# Autodesk Inventor assembly: Assembly1
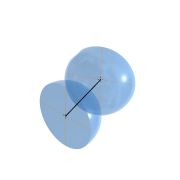
[picture p0: Inventor's stored thumbnail of the model, 180x180]
Saved by Autodesk Inventor 2020 (Build 240168000, 168)
## iProperties
Created: 2021-04-27
Part Number: Assembly1
Document SubType Name: Assembly
Designer: deox
Author: deox
## Documents named in this file (2)
- C:\Users\deox\Desktop\TCC\Inventor Files\Mechanism\Assembly1.iam
- C:\Users\deox\Desktop\TCC\Inventor Files\Mechanism\Ball.ipt
## Components (2 placed, 1 different names)
1. Ball:1 — Tangent:1, Angle:1
2. Ball:2 — Tangent:1, Angle:1
## Relationships (2: Tangent 1, Angle 1)
- Tangent:1: Ball:1 ↔ Ball:2
- Angle:1 (150 deg): Ball:1 ↔ Ball:2
